# Autodesk Inventor assembly: ST3215
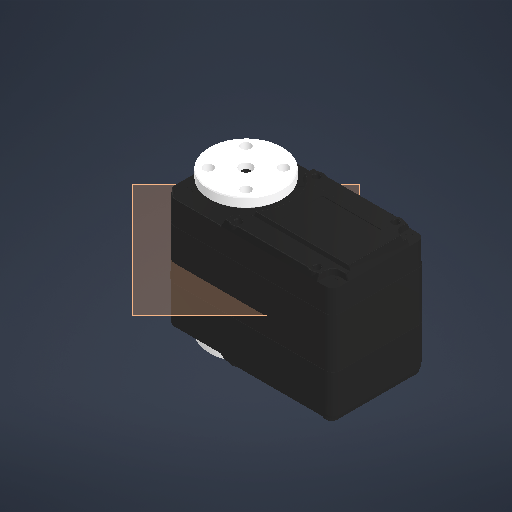
[picture p0: Inventor's stored thumbnail of the model, 512x512]
Saved by Autodesk Inventor 2026 (Build 300175000, 175)
## iProperties
Created: 2022-06-08
Part Number: ST3215
Document SubType Name: Assembly
Designer: paris
Sending System: Autodesk Translation Framework v11.7.0.108
Preprocessor: ST-DEVELOPER v19
Title: E:/ST3215/ST3215.step
## Documents named in this file (9)
- C:\Users\paris\OneDrive\Documents\GitHub\and-e\robot_manipulator_cad_files\Workspaces\Workspace\ST3215.iam
- C:\Users\paris\OneDrive\Documents\GitHub\and-e\robot_manipulator_cad_files\Workspaces\Workspace\ZK_122.ipt
- C:\Users\paris\OneDrive\Documents\GitHub\and-e\robot_manipulator_cad_files\Workspaces\Workspace\SG-ZIJI_15.ipt
- C:\Users\paris\OneDrive\Documents\GitHub\and-e\robot_manipulator_cad_files\Workspaces\Workspace\XG-ZIJI_16.ipt
- C:\Users\paris\OneDrive\Documents\GitHub\and-e\robot_manipulator_cad_files\Workspaces\Workspace\MOTOR-1723_3.ipt
- C:\Users\paris\OneDrive\Documents\GitHub\and-e\robot_manipulator_cad_files\Workspaces\Workspace\PCB-CHAZUO_92.ipt
- C:\Users\paris\OneDrive\Documents\GitHub\and-e\robot_manipulator_cad_files\Workspaces\Workspace\GE_27.ipt
- C:\Users\paris\OneDrive\Documents\GitHub\and-e\robot_manipulator_cad_files\Workspaces\Workspace\金属舵盘（驱动） v2.ipt
- C:\Users\paris\OneDrive\Documents\GitHub\and-e\robot_manipulator_cad_files\Workspaces\Workspace\金属舵盘（从动） v2.ipt
## Components (8 placed, 8 different names)
1. ZK_122:1
2. SG-ZIJI_15:1 — Mate:2
3. XG-ZIJI_16:1 — Mate:3, Flush:1
4. MOTOR-1723_3:1
5. PCB-CHAZUO_92:1
6. GE_27:1 — Mate:1
7. 金属舵盘（驱动） v2:1 — Mate:1, Mate:2, Mate:4, Mate:6, Mate:7, Symmetry:1
8. 金属舵盘（从动） v2:1 — Mate:3, Flush:1, Mate:4, Symmetry:1
## Relationships (11: Mate 8, Flush 1, Angle 1, Symmetry 1)
- Mate:1: GE_27:1 ↔ 金属舵盘（驱动） v2:1
- Mate:2: SG-ZIJI_15:1 ↔ 金属舵盘（驱动） v2:1
- Mate:3: XG-ZIJI_16:1 ↔ 金属舵盘（从动） v2:1
- Flush:1: XG-ZIJI_16:1 ↔ 金属舵盘（从动） v2:1
- Mate:4: 金属舵盘（驱动） v2:1 ↔ 金属舵盘（从动） v2:1
- Mate:6: 金属舵盘（驱动） v2:1
- Mate:7: 金属舵盘（驱动） v2:1
- Mate:8
- Mate:9
- Angle:1 (0 deg)
- Symmetry:1: 金属舵盘（驱动） v2:1 ↔ 金属舵盘（从动） v2:1
